# Autodesk Inventor assembly: ploter_1
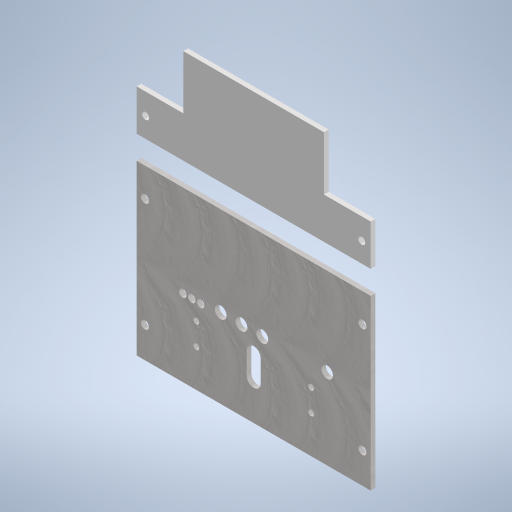
[picture p0: Inventor's stored thumbnail of the model, 512x512]
Saved by Autodesk Inventor 2023 (Build 270158000, 158)
## iProperties
Created: 2023-08-20
Part Number: ploter_1
Document SubType Name: Assembly
Designer: Kamil
Author: Kamil
## iProperties of the stored document MemberDocs/xAaaaqacaAaaaaaaaAaaaqi21Wa
Part Number: ploter_1
Document SubType Name: Zespół
Designer: Kamil
Author: Kamil
## Documents named in this file (4)
- C:\Users\Kamil\Desktop\MojeRoboty\Stefan\mechanics 2\ploter_1.iam
- C:\Users\Kamil\Desktop\MojeRoboty\Stefan\mechanics 2\tylna.ipt
- C:\Users\Kamil\Desktop\MojeRoboty\Stefan\mechanics 2\dach.ipt
- C:\Users\Kamil\Desktop\MojeRoboty\Stefan\mechanics 2\ploter_1_SUB.ipt
## Components (2 placed, 2 different names)
1. tylna:1 — Równoległe:1, Zestawiające:1, Równoległe:2
2. dach:1 — Równoległe:1, Zestawiające:1, Równoległe:2
## Relationships (3: Flush 2, Mate 1)
- Równoległe:1 [Flush]: tylna:1 ↔ dach:1
- Zestawiające:1 [Mate] (10 mm): tylna:1 ↔ dach:1
- Równoległe:2 [Flush]: tylna:1 ↔ dach:1
